# Autodesk Inventor assembly: Assembly of BOT!
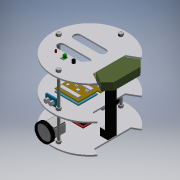
[picture p0: Inventor's stored thumbnail of the model, 180x180]
Saved by Autodesk Inventor 2018 (Build 220112000, 112)
## iProperties
Created: 2018-10-23
Part Number: Assembly of BOT!
Document SubType Name: Assembly
Designer: Melda
Author: Melda
## Documents named in this file (6)
- G:\Firefighter Parts\Assembly of BOT!.iam
- G:\Firefighter Parts\Bottom round.ipt
- G:\Firefighter Parts\Big screw thing.ipt
- G:\Firefighter Parts\Nut thing.ipt
- G:\Firefighter Parts\Middle round.ipt
- G:\Firefighter Parts\Top round.ipt
## Components (24 placed, 5 different names)
1. Bottom round:1 — Insert:1, Insert:2, Insert:3, Insert:7, Insert:8, Insert:9
2. Big screw thing:1 — Insert:6
3. Big screw thing:2 — Insert:5
4. Big screw thing:3 — Insert:4, Insert:10, Insert:11
5. Nut thing:1 — Insert:7
6. Nut thing:2 — Insert:12
7. Nut thing:3 — Insert:14
8. Nut thing:4 — Insert:13
9. Nut thing:5 — Insert:15
10. Nut thing:6 — Insert:16
11. Nut thing:7 — Insert:20
12. Nut thing:8 — Insert:19
13. Nut thing:9 — Insert:2, Insert:5
14. Nut thing:10 — Insert:3, Insert:6
15. Nut thing:11 — Insert:17
16. Nut thing:12 — Insert:23
17. Nut thing:13 — Insert:22
18. Nut thing:14 — Insert:21
19. Nut thing:15 — Insert:18
20. Nut thing:16 — Insert:9
21. Nut thing:17 — Insert:8
22. Nut thing:18 — Insert:1, Insert:4
23. Middle round:1 — Insert:10, Insert:12, Insert:13, Insert:14, Insert:18, Insert:19, Insert:20
24. Top round:1 — Insert:11, Insert:15, Insert:16, Insert:17, Insert:21, Insert:22, Insert:23
## Relationships (23: Insert 23)
- Insert:1: Bottom round:1 ↔ Nut thing:18
- Insert:2: Bottom round:1 ↔ Nut thing:9
- Insert:3: Bottom round:1 ↔ Nut thing:10
- Insert:4: Big screw thing:3 ↔ Nut thing:18
- Insert:5: Big screw thing:2 ↔ Nut thing:9
- Insert:6: Big screw thing:1 ↔ Nut thing:10
- Insert:7: Bottom round:1 ↔ Nut thing:1
- Insert:8: Bottom round:1 ↔ Nut thing:17
- Insert:9: Bottom round:1 ↔ Nut thing:16
- Insert:10 (120 mm): Big screw thing:3 ↔ Middle round:1
- Insert:11 (8 mm): Big screw thing:3 ↔ Top round:1
- Insert:12: Nut thing:2 ↔ Middle round:1
- Insert:13: Nut thing:4 ↔ Middle round:1
- Insert:14: Nut thing:3 ↔ Middle round:1
- Insert:15: Nut thing:5 ↔ Top round:1
- Insert:16: Nut thing:6 ↔ Top round:1
- Insert:17: Nut thing:11 ↔ Top round:1
- Insert:18: Nut thing:15 ↔ Middle round:1
- Insert:19: Nut thing:8 ↔ Middle round:1
- Insert:20: Nut thing:7 ↔ Middle round:1
- Insert:21: Nut thing:14 ↔ Top round:1
- Insert:22: Nut thing:13 ↔ Top round:1
- Insert:23: Nut thing:12 ↔ Top round:1
